# Autodesk Inventor assembly: Chassis
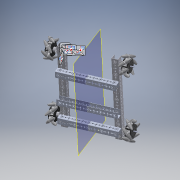
[picture p0: Inventor's stored thumbnail of the model, 180x180]
Saved by Autodesk Inventor 2018 (Build 220112000, 112)
## iProperties
Created: 2017-11-01
Part Number: Chassis
Document SubType Name: Assembly
Designer: Kitte
Author: Kitte
## Documents named in this file (20)
- C:\Users\Kitte\Documents\GitHub\7729-CAD\2017-18_CAD\Chassis.iam
- C:\Users\Kitte\Documents\Git\Robotics\lib\Tetrix\Structural_components\Channel 288mm.ipt
- C:\Users\Kitte\Documents\GitHub\7729-CAD\2017-18_CAD\Channel416mm_BearingHoles.ipt
- C:\Users\Kitte\Documents\GitHub\7729-CAD\lib\AndyMark\Misc\am-3377+6x12x4+Flanged+Bearing.ipt
- C:\Users\Kitte\Documents\GitHub\7729-CAD\lib\AndyMark\Misc\am-3226-100+6mm+D-Shaft+100mm.ipt
- C:\Users\Kitte\Documents\GitHub\7729-CAD\lib\Tetrix\Axels_hubs_and_collars\Motor Shaft (6mm) Hub.ipt
- C:\Users\Kitte\Documents\GitHub\7729-CAD\lib\Tetrix\Gears_and_sprockets\Gear 40 Tooth.ipt
- C:\Users\Kitte\Documents\GitHub\7729-CAD\lib\Tetrix\Gears_and_sprockets\am-2538 - 4 in mecanum left wheel.ipt
- C:\Users\Kitte\Documents\GitHub\7729-CAD\lib\Tetrix\Gears_and_sprockets\am-2538 - 4 in mecanum right wheel.ipt
- C:\Users\Kitte\Documents\GitHub\7729-CAD\lib\Tetrix\Axels_hubs_and_collars\Motor Shaft (6mm) Hub_CPY.ipt
- C:\Users\Kitte\Documents\GitHub\7729-CAD\lib\Tetrix\Gears_and_sprockets\Gear 40 Tooth_CPY.ipt
- C:\Users\Kitte\Documents\GitHub\7729-CAD\2017-18_CAD\Channel416mm_BearingHoles_MIR.ipt
- C:\Users\Kitte\Documents\GitHub\7729-CAD\lib\AndyMark\Misc\am-3377+6x12x4+Flanged+Bearing_MIR.ipt
- C:\Users\Kitte\Documents\GitHub\7729-CAD\lib\AndyMark\Misc\am-3226-100+6mm+D-Shaft+100mm_MIR.ipt
- C:\Users\Kitte\Documents\GitHub\7729-CAD\lib\Tetrix\Axels_hubs_and_collars\Motor Shaft (6mm) Hub_MIR.ipt
- C:\Users\Kitte\Documents\GitHub\7729-CAD\lib\Tetrix\Gears_and_sprockets\Gear 40 Tooth_MIR.ipt
- C:\Users\Kitte\Documents\GitHub\7729-CAD\lib\Tetrix\Gears_and_sprockets\am-2538 - 4 in mecanum left wheel_MIR.ipt
- C:\Users\Kitte\Documents\GitHub\7729-CAD\lib\Tetrix\Gears_and_sprockets\am-2538 - 4 in mecanum right wheel_MIR.ipt
- C:\Users\Kitte\Documents\GitHub\7729-CAD\lib\Tetrix\Axels_hubs_and_collars\Motor Shaft (6mm) Hub_CPY_MIR.ipt
- C:\Users\Kitte\Documents\GitHub\7729-CAD\lib\Tetrix\Gears_and_sprockets\Gear 40 Tooth_CPY_MIR.ipt
## Components (43 placed, 19 different names)
1. Channel 288mm:1 — Mate:10, Mate:11, Mate:66, Mate:67
2. Channel 288mm:2 — Mate:5, Mate:6, Mate:64
3. Channel 288mm:3 — Mate:7, Mate:8, Mate:26, Mate:65
4. Channel416mm_BearingHoles:1 — Mate:5, Mate:6, Mate:7, Mate:8, Mate:10, Mate:11, Insert:3, Insert:4, Insert:7, Insert:8, Angle:5
5. am-3377+6x12x4+Flanged+Bearing:1 — Insert:8, Mate:13, Mate:16, Mate:38
6. am-3377+6x12x4+Flanged+Bearing:2 — Insert:7, Mate:12, Mate:22, Mate:36
7. am-3377+6x12x4+Flanged+Bearing:5 — Insert:4, Mate:18, Mate:20
8. am-3377+6x12x4+Flanged+Bearing:6 — Insert:3, Mate:21, Mate:24
9. am-3226-100+6mm+D-Shaft+100mm:1 — Mate:12, Mate:21, Mate:23, Angle:3, Mate:25, Angle:4, Mate:35, Angle:6
10. am-3226-100+6mm+D-Shaft+100mm:4 — Mate:13, Mate:17, Mate:19, Angle:1, Angle:2, Mate:20, Mate:37, Angle:7, Angle:8
11. Motor Shaft (6mm) Hub:1 — Mate:24, Mate:25, Angle:4
12. Motor Shaft (6mm) Hub:4 — Mate:18, Mate:19, Angle:2
13. Motor Shaft (6mm) Hub:5 — Mate:16, Mate:17, Angle:1
14. Motor Shaft (6mm) Hub:8 — Mate:22, Mate:23, Angle:3
15. Motor Shaft (6mm) Hub:9 — Insert:9, Mate:27, Mate:28, Mate:29, Mate:30, Mate:35
16. Motor Shaft (6mm) Hub:10 — Mate:28, Mate:29, Mate:30, Angle:6, Insert:11, Mate:39
17. Gear 40 Tooth:1 — Insert:9, Mate:27, Mate:36
18. am-2538 - 4 in mecanum left wheel:1 — Insert:11, Mate:39
19. am-2538 - 4 in mecanum right wheel:1 — Insert:12, Angle:8
20. Motor Shaft (6mm) Hub_CPY:1 — Mate:31, Mate:32, Mate:33, Mate:34, Insert:10, Mate:37
21. Motor Shaft (6mm) Hub_CPY:2 — Mate:31, Mate:32, Mate:33, Angle:7, Insert:12
22. Gear 40 Tooth_CPY:1 — Mate:34, Insert:10, Mate:38
23. Channel416mm_BearingHoles_MIR:1 — Insert:13, Insert:14, Insert:15, Insert:16, Angle:13, Mate:64, Mate:65, Mate:66, Mate:67
24. am-3377+6x12x4+Flanged+Bearing_MIR:1 — Insert:13, Mate:43, Mate:49, Mate:62
25. am-3377+6x12x4+Flanged+Bearing_MIR:2 — Insert:14, Mate:41, Mate:51, Mate:56
26. am-3377+6x12x4+Flanged+Bearing_MIR:3 — Insert:15, Mate:42, Mate:47
27. am-3377+6x12x4+Flanged+Bearing_MIR:4 — Insert:16, Mate:40, Mate:45
28. am-3226-100+6mm+D-Shaft+100mm_MIR:1 — Mate:40, Mate:41, Angle:9, Mate:44, Angle:12, Mate:50, Mate:52, Angle:14
29. am-3226-100+6mm+D-Shaft+100mm_MIR:2 — Mate:42, Mate:43, Angle:10, Mate:46, Angle:11, Mate:48, Mate:58, Angle:15
30. Motor Shaft (6mm) Hub_MIR:1 — Angle:9, Mate:44, Mate:45
31. Motor Shaft (6mm) Hub_MIR:2 — Angle:10, Mate:46, Mate:47
32. Motor Shaft (6mm) Hub_MIR:3 — Angle:11, Mate:48, Mate:49
33. Motor Shaft (6mm) Hub_MIR:4 — Angle:12, Mate:50, Mate:51
34. Motor Shaft (6mm) Hub_MIR:5 — Mate:52, Mate:53, Mate:54, Mate:55, Mate:57, Insert:17
35. Motor Shaft (6mm) Hub_MIR:6 — Angle:14, Mate:53, Mate:54, Mate:55, Mate:69, Insert:20
36. Gear 40 Tooth_MIR:1 — Mate:56, Mate:57, Insert:17
37. am-2538 - 4 in mecanum left wheel_MIR:1
38. am-2538 - 4 in mecanum right wheel_MIR:1
39. Motor Shaft (6mm) Hub_CPY_MIR:1 — Mate:58, Mate:59, Mate:60, Mate:61, Insert:18, Mate:63
40. Motor Shaft (6mm) Hub_CPY_MIR:2 — Angle:15, Mate:59, Mate:60, Mate:61, Insert:19, Mate:68
41. Gear 40 Tooth_CPY_MIR:1 — Mate:62, Insert:18, Mate:63
42. am-2538 - 4 in mecanum right wheel:2 — Mate:69, Insert:20
43. am-2538 - 4 in mecanum left wheel:2 — Insert:19, Mate:68
## Relationships (93: Mate 62, Insert 16, Angle 15)
- Mate:5: Channel 288mm:2 ↔ Channel416mm_BearingHoles:1
- Mate:6: Channel 288mm:2 ↔ Channel416mm_BearingHoles:1
- Mate:7: Channel 288mm:3 ↔ Channel416mm_BearingHoles:1
- Mate:8: Channel 288mm:3 ↔ Channel416mm_BearingHoles:1
- Mate:10: Channel 288mm:1 ↔ Channel416mm_BearingHoles:1
- Mate:11: Channel 288mm:1 ↔ Channel416mm_BearingHoles:1
- Insert:3: Channel416mm_BearingHoles:1 ↔ am-3377+6x12x4+Flanged+Bearing:6
- Insert:4: Channel416mm_BearingHoles:1 ↔ am-3377+6x12x4+Flanged+Bearing:5
- Insert:7: Channel416mm_BearingHoles:1 ↔ am-3377+6x12x4+Flanged+Bearing:2
- Insert:8: Channel416mm_BearingHoles:1 ↔ am-3377+6x12x4+Flanged+Bearing:1
- Mate:12: am-3377+6x12x4+Flanged+Bearing:2 ↔ am-3226-100+6mm+D-Shaft+100mm:1
- Mate:13: am-3377+6x12x4+Flanged+Bearing:1 ↔ am-3226-100+6mm+D-Shaft+100mm:4
- Mate:16: am-3377+6x12x4+Flanged+Bearing:1 ↔ Motor Shaft (6mm) Hub:5
- Mate:17: am-3226-100+6mm+D-Shaft+100mm:4 ↔ Motor Shaft (6mm) Hub:5
- Mate:18: am-3377+6x12x4+Flanged+Bearing:5 ↔ Motor Shaft (6mm) Hub:4
- Mate:19: am-3226-100+6mm+D-Shaft+100mm:4 ↔ Motor Shaft (6mm) Hub:4
- Angle:1 (0 deg): am-3226-100+6mm+D-Shaft+100mm:4 ↔ Motor Shaft (6mm) Hub:5
- Angle:2 (0 deg): am-3226-100+6mm+D-Shaft+100mm:4 ↔ Motor Shaft (6mm) Hub:4
- Mate:20: am-3377+6x12x4+Flanged+Bearing:5 ↔ am-3226-100+6mm+D-Shaft+100mm:4
- Mate:21: am-3377+6x12x4+Flanged+Bearing:6 ↔ am-3226-100+6mm+D-Shaft+100mm:1
- Mate:22: am-3377+6x12x4+Flanged+Bearing:2 ↔ Motor Shaft (6mm) Hub:8
- Mate:23: am-3226-100+6mm+D-Shaft+100mm:1 ↔ Motor Shaft (6mm) Hub:8
- Angle:3 (0 deg): am-3226-100+6mm+D-Shaft+100mm:1 ↔ Motor Shaft (6mm) Hub:8
- Mate:24: am-3377+6x12x4+Flanged+Bearing:6 ↔ Motor Shaft (6mm) Hub:1
- Mate:25: am-3226-100+6mm+D-Shaft+100mm:1 ↔ Motor Shaft (6mm) Hub:1
- Angle:4 (0 deg): am-3226-100+6mm+D-Shaft+100mm:1 ↔ Motor Shaft (6mm) Hub:1
- Mate:26: Channel 288mm:3
- Angle:5 (0 deg): Channel416mm_BearingHoles:1
- Insert:9: Motor Shaft (6mm) Hub:9 ↔ Gear 40 Tooth:1
- Mate:27: Motor Shaft (6mm) Hub:9 ↔ Gear 40 Tooth:1
- Mate:28: Motor Shaft (6mm) Hub:9 ↔ Motor Shaft (6mm) Hub:10
- Mate:29: Motor Shaft (6mm) Hub:9 ↔ Motor Shaft (6mm) Hub:10
- Mate:30: Motor Shaft (6mm) Hub:9 ↔ Motor Shaft (6mm) Hub:10
- Mate:31: Motor Shaft (6mm) Hub_CPY:1 ↔ Motor Shaft (6mm) Hub_CPY:2
- Mate:32: Motor Shaft (6mm) Hub_CPY:1 ↔ Motor Shaft (6mm) Hub_CPY:2
- Mate:33: Motor Shaft (6mm) Hub_CPY:1 ↔ Motor Shaft (6mm) Hub_CPY:2
- Mate:34: Motor Shaft (6mm) Hub_CPY:1 ↔ Gear 40 Tooth_CPY:1
- Insert:10: Motor Shaft (6mm) Hub_CPY:1 ↔ Gear 40 Tooth_CPY:1
- Mate:35: am-3226-100+6mm+D-Shaft+100mm:1 ↔ Motor Shaft (6mm) Hub:9
- Mate:36 (2 mm): am-3377+6x12x4+Flanged+Bearing:2 ↔ Gear 40 Tooth:1
- Angle:6 (0 deg): am-3226-100+6mm+D-Shaft+100mm:1 ↔ Motor Shaft (6mm) Hub:10
- Mate:37: am-3226-100+6mm+D-Shaft+100mm:4 ↔ Motor Shaft (6mm) Hub_CPY:1
- Mate:38 (2 mm): am-3377+6x12x4+Flanged+Bearing:1 ↔ Gear 40 Tooth_CPY:1
- Angle:7 (0 deg): am-3226-100+6mm+D-Shaft+100mm:4 ↔ Motor Shaft (6mm) Hub_CPY:2
- Insert:11: Motor Shaft (6mm) Hub:10 ↔ am-2538 - 4 in mecanum left wheel:1
- Mate:39: Motor Shaft (6mm) Hub:10 ↔ am-2538 - 4 in mecanum left wheel:1
- Insert:12: am-2538 - 4 in mecanum right wheel:1 ↔ Motor Shaft (6mm) Hub_CPY:2
- Angle:8 (0 deg): am-3226-100+6mm+D-Shaft+100mm:4 ↔ am-2538 - 4 in mecanum right wheel:1
- Insert:13: Channel416mm_BearingHoles_MIR:1 ↔ am-3377+6x12x4+Flanged+Bearing_MIR:1
- Insert:14: Channel416mm_BearingHoles_MIR:1 ↔ am-3377+6x12x4+Flanged+Bearing_MIR:2
- Insert:15: Channel416mm_BearingHoles_MIR:1 ↔ am-3377+6x12x4+Flanged+Bearing_MIR:3
- Insert:16: Channel416mm_BearingHoles_MIR:1 ↔ am-3377+6x12x4+Flanged+Bearing_MIR:4
- Mate:40: am-3377+6x12x4+Flanged+Bearing_MIR:4 ↔ am-3226-100+6mm+D-Shaft+100mm_MIR:1
- Mate:41: am-3377+6x12x4+Flanged+Bearing_MIR:2 ↔ am-3226-100+6mm+D-Shaft+100mm_MIR:1
- Mate:42 (10 mm): am-3377+6x12x4+Flanged+Bearing_MIR:3 ↔ am-3226-100+6mm+D-Shaft+100mm_MIR:2
- Mate:43: am-3377+6x12x4+Flanged+Bearing_MIR:1 ↔ am-3226-100+6mm+D-Shaft+100mm_MIR:2
- Angle:9 (0 deg): am-3226-100+6mm+D-Shaft+100mm_MIR:1 ↔ Motor Shaft (6mm) Hub_MIR:1
- Mate:44: am-3226-100+6mm+D-Shaft+100mm_MIR:1 ↔ Motor Shaft (6mm) Hub_MIR:1
- Mate:45: am-3377+6x12x4+Flanged+Bearing_MIR:4 ↔ Motor Shaft (6mm) Hub_MIR:1
- Angle:10 (0 deg): am-3226-100+6mm+D-Shaft+100mm_MIR:2 ↔ Motor Shaft (6mm) Hub_MIR:2
- Mate:46: am-3226-100+6mm+D-Shaft+100mm_MIR:2 ↔ Motor Shaft (6mm) Hub_MIR:2
- Mate:47: am-3377+6x12x4+Flanged+Bearing_MIR:3 ↔ Motor Shaft (6mm) Hub_MIR:2
- Angle:11 (0 deg): am-3226-100+6mm+D-Shaft+100mm_MIR:2 ↔ Motor Shaft (6mm) Hub_MIR:3
- Mate:48: am-3226-100+6mm+D-Shaft+100mm_MIR:2 ↔ Motor Shaft (6mm) Hub_MIR:3
- Mate:49: am-3377+6x12x4+Flanged+Bearing_MIR:1 ↔ Motor Shaft (6mm) Hub_MIR:3
- Angle:12 (0 deg): am-3226-100+6mm+D-Shaft+100mm_MIR:1 ↔ Motor Shaft (6mm) Hub_MIR:4
- Mate:50: am-3226-100+6mm+D-Shaft+100mm_MIR:1 ↔ Motor Shaft (6mm) Hub_MIR:4
- Mate:51: am-3377+6x12x4+Flanged+Bearing_MIR:2 ↔ Motor Shaft (6mm) Hub_MIR:4
- Angle:13 (0 deg): Channel416mm_BearingHoles_MIR:1
- Mate:52: am-3226-100+6mm+D-Shaft+100mm_MIR:1 ↔ Motor Shaft (6mm) Hub_MIR:5
- Angle:14 (0 deg): am-3226-100+6mm+D-Shaft+100mm_MIR:1 ↔ Motor Shaft (6mm) Hub_MIR:6
- Mate:53: Motor Shaft (6mm) Hub_MIR:5 ↔ Motor Shaft (6mm) Hub_MIR:6
- Mate:54: Motor Shaft (6mm) Hub_MIR:5 ↔ Motor Shaft (6mm) Hub_MIR:6
- Mate:55: Motor Shaft (6mm) Hub_MIR:5 ↔ Motor Shaft (6mm) Hub_MIR:6
- Mate:56 (2 mm): am-3377+6x12x4+Flanged+Bearing_MIR:2 ↔ Gear 40 Tooth_MIR:1
- Mate:57: Motor Shaft (6mm) Hub_MIR:5 ↔ Gear 40 Tooth_MIR:1
- Insert:17: Motor Shaft (6mm) Hub_MIR:5 ↔ Gear 40 Tooth_MIR:1
- Mate:58: am-3226-100+6mm+D-Shaft+100mm_MIR:2 ↔ Motor Shaft (6mm) Hub_CPY_MIR:1
- Angle:15 (0 deg): am-3226-100+6mm+D-Shaft+100mm_MIR:2 ↔ Motor Shaft (6mm) Hub_CPY_MIR:2
- Mate:59: Motor Shaft (6mm) Hub_CPY_MIR:1 ↔ Motor Shaft (6mm) Hub_CPY_MIR:2
- Mate:60: Motor Shaft (6mm) Hub_CPY_MIR:1 ↔ Motor Shaft (6mm) Hub_CPY_MIR:2
- Mate:61: Motor Shaft (6mm) Hub_CPY_MIR:1 ↔ Motor Shaft (6mm) Hub_CPY_MIR:2
- Mate:62 (2 mm): am-3377+6x12x4+Flanged+Bearing_MIR:1 ↔ Gear 40 Tooth_CPY_MIR:1
- Insert:18: Motor Shaft (6mm) Hub_CPY_MIR:1 ↔ Gear 40 Tooth_CPY_MIR:1
- Mate:63: Motor Shaft (6mm) Hub_CPY_MIR:1 ↔ Gear 40 Tooth_CPY_MIR:1
- Mate:64: Channel 288mm:2 ↔ Channel416mm_BearingHoles_MIR:1
- Mate:65: Channel 288mm:3 ↔ Channel416mm_BearingHoles_MIR:1
- Mate:66: Channel 288mm:1 ↔ Channel416mm_BearingHoles_MIR:1
- Mate:67: Channel 288mm:1 ↔ Channel416mm_BearingHoles_MIR:1
- Insert:19: Motor Shaft (6mm) Hub_CPY_MIR:2 ↔ am-2538 - 4 in mecanum left wheel:2
- Mate:68: Motor Shaft (6mm) Hub_CPY_MIR:2 ↔ am-2538 - 4 in mecanum left wheel:2
- Mate:69: Motor Shaft (6mm) Hub_MIR:6 ↔ am-2538 - 4 in mecanum right wheel:2
- Insert:20: Motor Shaft (6mm) Hub_MIR:6 ↔ am-2538 - 4 in mecanum right wheel:2
